# Autodesk Inventor assembly: attocube_stack_ohne_heater_ohne_boden
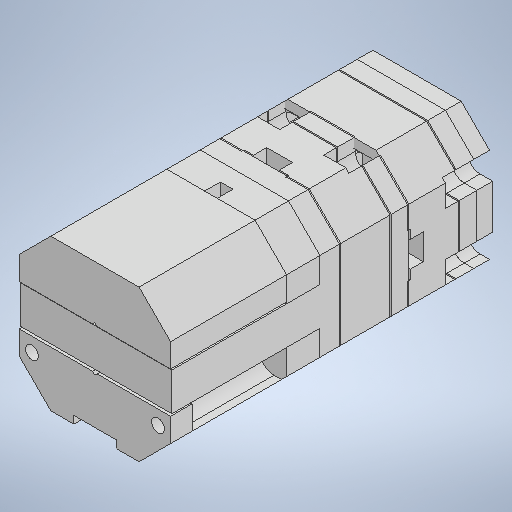
[picture p0: Inventor's stored thumbnail of the model, 512x512]
Saved by Autodesk Inventor 2026.1 (Build 301233000, 233)
## iProperties
Created: 2018-09-11
Part Number: attocube_stack_ohne_heater_ohne_boden
Document SubType Name: Assembly
Designer: Q
Author: Q
## Documents named in this file (4)
- C:\Users\user\Desktop\setup_inventor_2025\attocube\attocube_stack_ohne_heater_ohne_boden.iam
- C:\Users\user\Desktop\setup_inventor_2025\attocube\ANPx101_RES.iam
- C:\Users\user\Desktop\setup_inventor_2025\attocube\ANPz102_RES.ipt
- C:\Users\user\Desktop\setup_inventor_2025\attocube\ANPx101res_2_5mm_spacer.ipt
## Components (4 placed, 3 different names)
1. ANPz102_RES:1 — Mate:2, Flush:3, Flush:4
2. ANPx101_RES:1 [sub-assembly] — Mate:2, Flush:3, Flush:4, Mate:3, Flush:5, Flush:6
3. ANPx101_RES:2 [sub-assembly] — Mate:3, Flush:5, Flush:6, Mate:4, Mate:5, Mate:6
4. ANPx101res_2_5mm_spacer:1 — Mate:4, Mate:5, Mate:6
## Relationships (9: Mate 5, Flush 4)
- Mate:2: ANPz102_RES:1 ↔ ANPx101_RES:1
- Flush:3: ANPz102_RES:1 ↔ ANPx101_RES:1
- Flush:4: ANPz102_RES:1 ↔ ANPx101_RES:1
- Mate:3: ANPx101_RES:1 ↔ ANPx101_RES:2
- Flush:5: ANPx101_RES:1 ↔ ANPx101_RES:2
- Flush:6: ANPx101_RES:1 ↔ ANPx101_RES:2
- Mate:4: ANPx101_RES:2 ↔ ANPx101res_2_5mm_spacer:1
- Mate:5: ANPx101_RES:2 ↔ ANPx101res_2_5mm_spacer:1
- Mate:6: ANPx101_RES:2 ↔ ANPx101res_2_5mm_spacer:1
